# Autodesk Inventor assembly: KarMerev
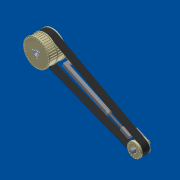
[picture p0: Inventor's stored thumbnail of the model, 180x180]
Saved by Autodesk Inventor 2015 SP1 (Build 190203100, 203)
## iProperties
Created: 2015-02-26
Part Number: KarMerev
Document SubType Name: Assembly
Designer: laca
Mass: 1010.29 g
Surface Area: 2601.12 cm^2
Volume: 909.657 cm^3
Density: 1.11063 g/cm^3
Author: laca
## Documents named in this file (9)
- C:\Users\laca\Desktop\Allamvizsga\Invntor\RobotMechanikaForMAtlabVer2\KarMerev.iam
- C:\Users\laca\Desktop\Allamvizsga\Invntor\RobotMechanikaForMAtlabVer2\NagyKerek.ipt
- C:\Users\laca\Desktop\Allamvizsga\Invntor\RobotMechanikaForMAtlabVer2\KissKerek.ipt
- C:\Users\laca\Desktop\Allamvizsga\Invntor\RobotMechanikaForMAtlabVer2\6001 BEARING.iam
- C:\Users\laca\Desktop\Allamvizsga\Invntor\RobotMechanikaForMAtlabVer2\Alkar.ipt
- C:\Users\laca\Desktop\Allamvizsga\Invntor\RobotMechanikaForMAtlabVer2\Felkar.ipt
- C:\Users\laca\Desktop\Allamvizsga\Invntor\RobotMechanikaForMAtlabVer2\KisTenge.ipt
- C:\Users\laca\Desktop\Allamvizsga\Invntor\RobotMechanikaForMAtlabVer2\SpanoloAnya.ipt
- C:\Users\laca\Desktop\Allamvizsga\Invntor\RobotMechanikaForMAtlabVer2\Szij.ipt
## Components (12 placed, 8 different names)
1. NagyKerek:1
2. KissKerek:1
3. 6001 BEARING:1 [sub-assembly]
4. 6001 BEARING:2 [sub-assembly] — Insert:2
5. 6001 BEARING:3 [sub-assembly]
6. 6001 BEARING:4 [sub-assembly]
7. Alkar:1 — Insert:2
8. Felkar:1 — Insert:1
9. KisTenge:1 — Insert:1
10. SpanoloAnya:1
11. SpanoloAnya:2
12. Szij:1
## Relationships (15: WeldJoint 5, Mate 4, RevoluteJoint 3, Insert 2, CylindricalJoint 1)
- [WeldJoint]: NagyKerek:1 ↔ 6001 BEARING:1
- [WeldJoint]: NagyKerek:1 ↔ 6001 BEARING:2
- [WeldJoint]: KissKerek:1 ↔ 6001 BEARING:4
- [WeldJoint]: KissKerek:1 ↔ 6001 BEARING:3
- [WeldJoint]: 6001 BEARING:4 ↔ KisTenge:1
- [RevoluteJoint]: 6001 BEARING:3 ↔ SpanoloAnya:2
- [RevoluteJoint]: NagyKerek:1 ↔ Szij:1
- [Mate]: Alkar:1 ↔ Felkar:1
- [Mate]: Alkar:1 ↔ Felkar:1
- Insert:1 (-1 mm): Felkar:1 ↔ KisTenge:1
- [RevoluteJoint]: KissKerek:1 ↔ Szij:1
- [Mate]: Alkar:1 ↔ SpanoloAnya:1
- [CylindricalJoint]: Felkar:1 ↔ SpanoloAnya:1
- [Mate]: Alkar:1 ↔ Felkar:1
- Insert:2 (3 mm): 6001 BEARING:2 ↔ Alkar:1
## Named parameters: d8_d20 = 0 mm
